# Autodesk Inventor assembly: 60645K311
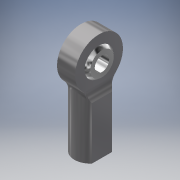
[picture p0: Inventor's stored thumbnail of the model, 180x180]
Saved by Autodesk Inventor 2016 SP2 (Build 200236200, 236)
## iProperties
Created: 2017-02-16
Part Number: 60645K311
Document SubType Name: Assembly
Designer: 589013
Description: 10-32 Super Duty Linkage
Mass: 15.5192 g
Surface Area: 21.6994 cm^2
Volume: 1.9399 cm^3
Density: 8 g/cm^3
Author: smiku
Title: 60645K311
## Documents named in this file (3)
- C:\Users\smiku\GrabCAD\Power Hawks CAD\ServoCity Resources\Structure\10-32SuperDutyLinkage-1111-2017.iam
- C:\Users\smiku\GrabCAD\Power Hawks CAD\ServoCity Resources\Structure\10-32SuperDutyLinkage\10-32SuperDutyLinkage(Housing)-1111-2017.ipt
- C:\Users\smiku\GrabCAD\Power Hawks CAD\ServoCity Resources\Structure\10-32SuperDutyLinkage\10-32SuperDutyLinkage(Ball)-1111-2017.ipt
## Components (2 placed, 2 different names)
1. 10-32SuperDutyLinkage(Housing)-1111-2017:1 — Flush:1, Ball:1
2. 10-32SuperDutyLinkage(Ball)-1111-2017:1 — Flush:1, Ball:1
## Relationships (2: Flush 1, BallJoint 1)
- Flush:1: 10-32SuperDutyLinkage(Housing)-1111-2017:1 ↔ 10-32SuperDutyLinkage(Ball)-1111-2017:1
- Ball:1: 10-32SuperDutyLinkage(Housing)-1111-2017:1 ↔ 10-32SuperDutyLinkage(Ball)-1111-2017:1
